# Autodesk Inventor assembly: X Axis (1)
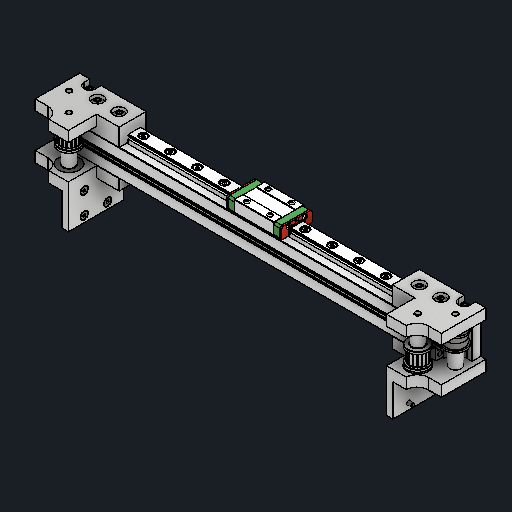
[picture p0: Inventor's stored thumbnail of the model, 512x512]
Saved by Autodesk Inventor 2026.1 (Build 301233020, 233B)
## iProperties
Created: 2025-05-23
Part Number: X Axis (1)
Document SubType Name: Assembly
Designer: Joshua Eah
Author: Joshua Eah
## Documents named in this file (5)
- C:\Users\JoshuaEah\Documents\GitHub\Voron-0\CAD\Tulip - Machined Parts\Tulip Mod Master\X Axis.iam
- C:\Users\JoshuaEah\Documents\GitHub\Voron-0\CAD\Tulip - Machined Parts\Tulip Mod Master\MGN7H.iam
- C:\Users\JoshuaEah\Documents\GitHub\Voron-0\CAD\Tulip - Machined Parts\XY Joints\XY Joint Left\XY Joint Left (Tulip).iam
- C:\Users\JoshuaEah\Documents\GitHub\Voron-0\CAD\Tulip - Machined Parts\XY Joints\XY Joint Right\XY Joint Right (Tulip).iam
- C:\Users\JoshuaEah\Documents\GitHub\Voron-0\CAD\Tulip - Machined Parts\Tulip Mod Master\1515 200mm - A (1) (1).ipt
## Components (4 placed, 4 different names)
1. XY Joint Left (Tulip):1 [sub-assembly] — Mate:2
2. XY Joint Right (Tulip):1 [sub-assembly] — Mate:3, Mate:4, Flush:2
3. MGN7H:1 [sub-assembly] — Mate:2, Mate:4
4. 1515 200mm - A (1) (1):1 — Mate:3, Flush:2
## Relationships (6: Mate 4, Flush 2)
- [Mate]: XY Joint Left (Tulip):1 ↔ 1515 200mm - A (1) (1):1
- [Flush]: XY Joint Left (Tulip):1 ↔ 1515 200mm - A (1) (1):1
- Mate:2 (1 mm): XY Joint Left (Tulip):1 ↔ MGN7H:1
- Mate:3: XY Joint Right (Tulip):1 ↔ 1515 200mm - A (1) (1):1
- Mate:4 (1 mm): XY Joint Right (Tulip):1 ↔ MGN7H:1
- Flush:2: XY Joint Right (Tulip):1 ↔ 1515 200mm - A (1) (1):1
